# Autodesk Inventor assembly: motor_set_left
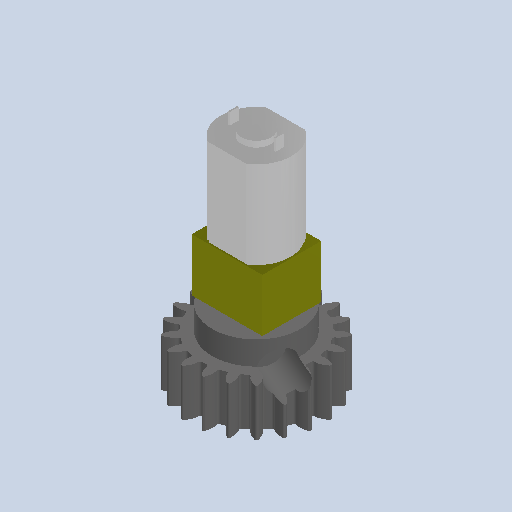
[picture p0: Inventor's stored thumbnail of the model, 512x512]
Saved by Autodesk Inventor 2024.1 (Build 281209000, 209)
## iProperties
Created: 2025-01-18
Part Number: motor_set_left
Document SubType Name: Assembly
Designer: hibik
Author: hibik
## Documents named in this file (5)
- C:\Users\hibik\Documents\Robomech\RESCUE\ORCA\hard\fork\left\motor_set_left.iam
- C:\Users\hibik\Documents\Robomech\RESCUE\ORCA\hard\fork\left\motor_6V_60RPM_left.ipt
- C:\Users\hibik\Documents\Robomech\RESCUE\ORCA\hard\fork\left\screw_bearing_setter_left.ipt
- C:\Users\hibik\Documents\Robomech\RESCUE\ORCA\hard\fork\left\screw_gear_under_left.ipt
- C:\Users\hibik\Documents\Robomech\RESCUE\ORCA\hard\fork\left\bearing_6_10_3_left.ipt
## Components (4 placed, 4 different names)
1. motor_6V_60RPM_left:1 — 挿入:3
2. screw_bearing_setter_left:1 — 挿入:3, 挿入:2
3. screw_gear_under_left:1 — 挿入:1
4. bearing_6_10_3_left:1 — 挿入:2, 挿入:1
## Relationships (3: Insert 3)
- 挿入:3 [Insert]: motor_6V_60RPM_left:1 ↔ screw_bearing_setter_left:1
- 挿入:2 [Insert]: screw_bearing_setter_left:1 ↔ bearing_6_10_3_left:1
- 挿入:1 [Insert]: screw_gear_under_left:1 ↔ bearing_6_10_3_left:1
